# Autodesk Inventor assembly: robotshow
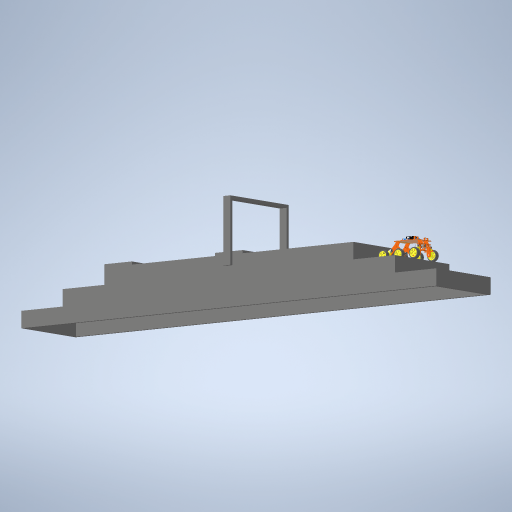
[picture p0: Inventor's stored thumbnail of the model, 512x512]
Saved by Autodesk Inventor 2023.2 (Build 272271000, 271)
## iProperties
Created: 2022-11-26
Part Number: robotshow
Document SubType Name: Assembly
Designer: omrfrkmll
Author: omrfrkmll
## Documents named in this file (27)
- C:\Users\omr_f\Desktop\mechanism design project\robotshow.iam
- C:\Users\omr_f\Desktop\mechanism design project\6v dc torque motor.iam
- C:\Users\omr_f\Desktop\mechanism design project\Wheel D65x25.ipt
- C:\Users\omr_f\Desktop\mechanism design project\robotbase.ipt
- C:\Users\omr_f\Desktop\mechanism design project\sol arka bacak.ipt
- C:\Users\omr_f\Desktop\mechanism design project\sağ arka bacak.ipt
- C:\Users\omr_f\Desktop\mechanism design project\ön sol bacak.ipt
- C:\Users\omr_f\Desktop\mechanism design project\ön sol bacak_MIR.ipt
- C:\Users\omr_f\Desktop\mechanism design project\bişeyleramabendeisimveremedim.ipt
- C:\Users\omr_f\Desktop\mechanism design project\pin.ipt
- C:\Users\omr_f\Desktop\mechanism design project\pintutucu.ipt
- C:\Users\omr_f\Desktop\mechanism design project\pintutucu_MIR.ipt
- C:\Users\omr_f\Desktop\mechanism design project\bilmemç.ipt
- C:\Users\omr_f\Desktop\mechanism design project\Moteur - Moteur.ipt
- C:\Users\omr_f\Desktop\mechanism design project\screw.ipt
- C:\Users\omr_f\Desktop\mechanism design project\dişli.ipt
- C:\Users\omr_f\Desktop\mechanism design project\somun.ipt
- C:\Users\omr_f\Desktop\mechanism design project\benniyebuçüklerinsiminibilmiyorum.ipt
- C:\Users\omr_f\Desktop\mechanism design project\platform.ipt
- C:\Users\omr_f\Desktop\mechanism design project\ufakpin.ipt
- C:\Users\omr_f\Desktop\mechanism design project\rockerbogieçükü.ipt
- C:\Users\omr_f\Desktop\mechanism design project\6v dc torque motor_MIR.iam
- C:\Users\omr_f\Desktop\mechanism design project\Wheel D65x25_MIR.ipt
- C:\Users\omr_f\Desktop\mechanism design project\rockerbogieçükü_MIR.ipt
- C:\Users\omr_f\Desktop\mechanism design project\çıkçık.ipt
- C:\Users\omr_f\Desktop\mechanism design project\çıkçıkkarşılıkk.ipt
- C:\Users\omr_f\Desktop\mechanism design project\L298N Driver DC Motor.ipt
## Components (39 placed, 26 different names)
1. robotbase:1 — Mate:39, Mate:40, Mate:41, Mate:42, Mate:44, Mate:53, Mate:54, Mate:55, Mate:56, Mate:57, Mate:58, Mate:59, Mate:113, Mate:143, Mate:144, Mate:145
2. sağ arka bacak:1 — Mate:41, Mate:42, Mate:44, Mate:134, Mate:136
3. sol arka bacak:1 — Mate:39, Mate:40, Mate:53, Mate:114, Mate:115, Mate:135, Mate:139
4. 6v dc torque motor:5 [sub-assembly] — Mate:116, Mate:117, Mate:118
5. Wheel D65x25:5
6. ön sol bacak:1 — Mate:54, Mate:55, Mate:56
7. ön sol bacak_MIR:1 — Mate:57, Mate:58, Mate:59, Mate:66, Mate:67, Mate:68
8. 6v dc torque motor:6 [sub-assembly] — Mate:75, Mate:77, Mate:78, Mate:110, Mate:111
9. Wheel D65x25:6
10. bişeyleramabendeisimveremedim:1 — Mate:66, Mate:67, Mate:68, Mate:69, Mate:70, Mate:79, Mate:80, Mate:92, Mate:93, Mate:94, Angle:1, Mate:100
11. pin:1 — Mate:69, Mate:70, Mate:72, Mate:74, Mate:76
12. pintutucu:1 — Mate:72, Mate:74, Mate:75, Mate:76, Mate:77, Mate:78, Mate:85, Mate:110, Mate:111
13. pintutucu_MIR:1 — Mate:81, Mate:82, Mate:83, Mate:84, Mate:89, Mate:90, Mate:91
14. pin:2 — Mate:79, Mate:80, Mate:81, Mate:82, Mate:83
15. bilmemç:1 — Mate:84, Mate:85, Mate:142
16. 6v dc torque motor:7 [sub-assembly] — Mate:89, Mate:90, Mate:91
17. Wheel D65x25:7
18. Moteur - Moteur:1 — Mate:92, Mate:93, Mate:95, Mate:99
19. screw:1 — Mate:97, Mate:98, Mate:100, Mate:101
20. dişli:1 — Mate:97, Mate:98, Mate:99
21. somun:1 — Mate:101, Mate:102, Mate:103
22. benniyebuçüklerinsiminibilmiyorum:1 — Mate:102, Mate:103, Mate:141
23. platform:1 — Mate:113
24. ufakpin:1 — Mate:141, Mate:142
25. rockerbogieçükü:1 — Mate:114, Mate:115, Mate:116, Mate:117, Mate:118, Mate:121, Mate:122, Mate:123, Mate:135, Mate:137, Mate:138
26. 6v dc torque motor:8 [sub-assembly] — Mate:121, Mate:122, Mate:123
27. Wheel D65x25:8
28. 6v dc torque motor_MIR:1 [sub-assembly] — Mate:124, Mate:125, Mate:126, Mate:127, Mate:128
29. Wheel D65x25_MIR:1 — Mate:124, Mate:125
30. rockerbogieçükü_MIR:1 — Mate:126, Mate:127, Mate:128, Mate:129, Mate:130, Mate:131, Mate:134, Mate:136, Mate:146, Mate:147, Mate:148
31. 6v dc torque motor_MIR:2 [sub-assembly] — Mate:129, Mate:130, Mate:131, Mate:132, Mate:133
32. Wheel D65x25_MIR:2 — Mate:132, Mate:133
33. çıkçık:1 — Mate:137, Mate:138, Mate:140
34. çıkçıkkarşılıkk:1 — Mate:139, Mate:140
35. L298N Driver DC Motor:1 — Mate:145
36. L298N Driver DC Motor:2 — Mate:144
37. L298N Driver DC Motor:3 — Mate:143
38. çıkçık:2 — Mate:146, Mate:148, Mate:149
39. çıkçıkkarşılıkk:2 — Mate:147, Mate:149
## Relationships (90: Mate 89, Angle 1)
- Mate:39: robotbase:1 ↔ sol arka bacak:1
- Mate:40: robotbase:1 ↔ sol arka bacak:1
- Mate:41: robotbase:1 ↔ sağ arka bacak:1
- Mate:42: robotbase:1 ↔ sağ arka bacak:1
- Mate:44: robotbase:1 ↔ sağ arka bacak:1
- [Mate]: 6v dc torque motor:5 ↔ Wheel D65x25:5
- [Mate]: 6v dc torque motor:5 ↔ Wheel D65x25:5
- Mate:53: robotbase:1 ↔ sol arka bacak:1
- Mate:54: robotbase:1 ↔ ön sol bacak:1
- Mate:55: robotbase:1 ↔ ön sol bacak:1
- Mate:56: robotbase:1 ↔ ön sol bacak:1
- Mate:57: robotbase:1 ↔ ön sol bacak_MIR:1
- Mate:58: robotbase:1 ↔ ön sol bacak_MIR:1
- Mate:59: robotbase:1 ↔ ön sol bacak_MIR:1
- [Mate]: 6v dc torque motor:6 ↔ Wheel D65x25:6
- [Mate]: 6v dc torque motor:6 ↔ Wheel D65x25:6
- Mate:66: ön sol bacak_MIR:1 ↔ bişeyleramabendeisimveremedim:1
- Mate:67: ön sol bacak_MIR:1 ↔ bişeyleramabendeisimveremedim:1
- Mate:68: ön sol bacak_MIR:1 ↔ bişeyleramabendeisimveremedim:1
- Mate:69: bişeyleramabendeisimveremedim:1 ↔ pin:1
- Mate:70: bişeyleramabendeisimveremedim:1 ↔ pin:1
- Mate:72: pin:1 ↔ pintutucu:1
- Mate:74: pin:1 ↔ pintutucu:1
- Mate:75: 6v dc torque motor:6 ↔ pintutucu:1
- Mate:76: pin:1 ↔ pintutucu:1
- Mate:77: 6v dc torque motor:6 ↔ pintutucu:1
- Mate:78: 6v dc torque motor:6 ↔ pintutucu:1
- Mate:79: bişeyleramabendeisimveremedim:1 ↔ pin:2
- Mate:80: bişeyleramabendeisimveremedim:1 ↔ pin:2
- Mate:81: pintutucu_MIR:1 ↔ pin:2
- Mate:82: pintutucu_MIR:1 ↔ pin:2
- Mate:83: pintutucu_MIR:1 ↔ pin:2
- Mate:84: pintutucu_MIR:1 ↔ bilmemç:1
- Mate:85: pintutucu:1 ↔ bilmemç:1
- [Mate]: 6v dc torque motor:7 ↔ Wheel D65x25:7
- [Mate]: 6v dc torque motor:7 ↔ Wheel D65x25:7
- Mate:89: pintutucu_MIR:1 ↔ 6v dc torque motor:7
- Mate:90: pintutucu_MIR:1 ↔ 6v dc torque motor:7
- Mate:91: pintutucu_MIR:1 ↔ 6v dc torque motor:7
- Mate:92: bişeyleramabendeisimveremedim:1 ↔ Moteur - Moteur:1
- Mate:93: bişeyleramabendeisimveremedim:1 ↔ Moteur - Moteur:1
- Mate:94: bişeyleramabendeisimveremedim:1
- Angle:1 (0 deg): bişeyleramabendeisimveremedim:1
- Mate:95: Moteur - Moteur:1
- Mate:97: screw:1 ↔ dişli:1
- Mate:98: screw:1 ↔ dişli:1
- Mate:99 (7 mm): Moteur - Moteur:1 ↔ dişli:1
- Mate:100: bişeyleramabendeisimveremedim:1 ↔ screw:1
- Mate:101: screw:1 ↔ somun:1
- Mate:102: somun:1 ↔ benniyebuçüklerinsiminibilmiyorum:1
- Mate:103: somun:1 ↔ benniyebuçüklerinsiminibilmiyorum:1
- Mate:110: 6v dc torque motor:6 ↔ pintutucu:1
- Mate:111: 6v dc torque motor:6 ↔ pintutucu:1
- Mate:113 (116 mm): robotbase:1 ↔ platform:1
- Mate:114: sol arka bacak:1 ↔ rockerbogieçükü:1
- Mate:115: sol arka bacak:1 ↔ rockerbogieçükü:1
- Mate:116: 6v dc torque motor:5 ↔ rockerbogieçükü:1
- Mate:117: 6v dc torque motor:5 ↔ rockerbogieçükü:1
- Mate:118: 6v dc torque motor:5 ↔ rockerbogieçükü:1
- [Mate]: 6v dc torque motor:8 ↔ Wheel D65x25:8
- [Mate]: 6v dc torque motor:8 ↔ Wheel D65x25:8
- Mate:121: rockerbogieçükü:1 ↔ 6v dc torque motor:8
- Mate:122: rockerbogieçükü:1 ↔ 6v dc torque motor:8
- Mate:123: rockerbogieçükü:1 ↔ 6v dc torque motor:8
- Mate:124: 6v dc torque motor_MIR:1 ↔ Wheel D65x25_MIR:1
- Mate:125: 6v dc torque motor_MIR:1 ↔ Wheel D65x25_MIR:1
- Mate:126: 6v dc torque motor_MIR:1 ↔ rockerbogieçükü_MIR:1
- Mate:127: 6v dc torque motor_MIR:1 ↔ rockerbogieçükü_MIR:1
- Mate:128: 6v dc torque motor_MIR:1 ↔ rockerbogieçükü_MIR:1
- Mate:129: rockerbogieçükü_MIR:1 ↔ 6v dc torque motor_MIR:2
- Mate:130: rockerbogieçükü_MIR:1 ↔ 6v dc torque motor_MIR:2
- Mate:131: rockerbogieçükü_MIR:1 ↔ 6v dc torque motor_MIR:2
- Mate:132: 6v dc torque motor_MIR:2 ↔ Wheel D65x25_MIR:2
- Mate:133: 6v dc torque motor_MIR:2 ↔ Wheel D65x25_MIR:2
- Mate:134: sağ arka bacak:1 ↔ rockerbogieçükü_MIR:1
- Mate:135: sol arka bacak:1 ↔ rockerbogieçükü:1
- Mate:136: sağ arka bacak:1 ↔ rockerbogieçükü_MIR:1
- Mate:137: rockerbogieçükü:1 ↔ çıkçık:1
- Mate:138: rockerbogieçükü:1 ↔ çıkçık:1
- Mate:139: sol arka bacak:1 ↔ çıkçıkkarşılıkk:1
- Mate:140: çıkçık:1 ↔ çıkçıkkarşılıkk:1
- Mate:141: benniyebuçüklerinsiminibilmiyorum:1 ↔ ufakpin:1
- Mate:142: bilmemç:1 ↔ ufakpin:1
- Mate:143: robotbase:1 ↔ L298N Driver DC Motor:3
- Mate:144: robotbase:1 ↔ L298N Driver DC Motor:2
- Mate:145: robotbase:1 ↔ L298N Driver DC Motor:1
- Mate:146: rockerbogieçükü_MIR:1 ↔ çıkçık:2
- Mate:147: rockerbogieçükü_MIR:1 ↔ çıkçıkkarşılıkk:2
- Mate:148: rockerbogieçükü_MIR:1 ↔ çıkçık:2
- Mate:149: çıkçık:2 ↔ çıkçıkkarşılıkk:2
## Named parameters: d59_d45 = 0 mm, d60_d46 = 0 mm, d77_d45 = 0 mm, d78_d46 = 0 mm, d100_d59_d45 = 0 mm, d101_d60_d46 = 0 mm, d156_d59_d45 = 0 mm, d157_d60_d46 = 0 mm
